# Autodesk Inventor assembly: Gearbox
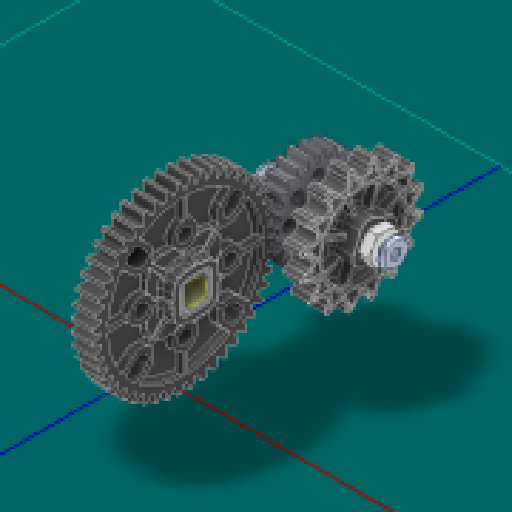
[picture p0: Inventor's stored thumbnail of the model, 512x512]
Saved by Autodesk Inventor 2025 (Build 290162000, 162)
## iProperties
Created: 2024-10-21
Part Number: Gearbox
Document SubType Name: Assembly
Designer: averey
Author: averey
## Documents named in this file (12)
- C:\Users\avere\VEX\High Stakes\CAD\V2\Intake\Gearbox.iam
- Gearbox Left.iam
- C:\Users\avere\VEX\High Stakes\CAD\ROBOPROS-CAD-Inventor\Motion\Sprockets\6P Sprocket\6P 16T Sprocket, No Insert.iam
- C:\Users\avere\VEX\High Stakes\CAD\V2\Intake\Custom Parts\Gearbox Gusset.ipt
- C:\Users\avere\VEX\High Stakes\CAD\ROBOPROS-CAD-Inventor\Structure\Hardware\Nut Nylon\Nut Nylon - White.ipt
- C:\Users\avere\VEX\High Stakes\CAD\ROBOPROS-CAD-Inventor\Structure\Hardware\Nut Nylon.ipt
- C:\Users\avere\VEX\High Stakes\CAD\ROBOPROS-CAD-Inventor\Structure\Hardware\Nut Thin Nylock.ipt
- C:\Users\avere\VEX\High Stakes\CAD\ROBOPROS-CAD-Inventor\Structure\Hardware\Screw Steel - Star\SScrew Star Smooth 1.500.ipt
- C:\Users\avere\VEX\High Stakes\CAD\ROBOPROS-CAD-Inventor\Structure\Hardware\Screw Steel - Star.ipt
- C:\Users\avere\VEX\High Stakes\CAD\ROBOPROS-CAD-Inventor\Motion\Sprockets\6P Sprocket.iam
- C:\Users\avere\VEX\High Stakes\CAD\ROBOPROS-CAD-Inventor\Modified Parts\Half Cut HS 24T Gear, No Insert.ipt
- C:\Users\avere\VEX\High Stakes\CAD\ROBOPROS-CAD-Inventor\Modified Parts\Equal Half Cut HS 48T Gear, No Insert.ipt
## Components (7 placed, 7 different names)
1. 6P 16T Sprocket, No Insert:1 [sub-assembly] — Insert:4
2. Gearbox Gusset:1 — Mate:2, Mate:3, Mate:4, Insert:5, Insert:9, Insert:10
3. Nut Nylon - White:1 — Insert:4, Insert:6
4. Nut Thin Nylock:1 — Insert:5
5. SScrew Star Smooth 1.500:1 — Insert:6
6. Half Cut HS 24T Gear, No Insert:1 — Insert:9
7. Equal Half Cut HS 48T Gear, No Insert:1 — Insert:10
## Relationships (8: Insert 5, Mate 3)
- Mate:2: Gearbox Gusset:1
- Mate:3: Gearbox Gusset:1
- Mate:4: Gearbox Gusset:1
- Insert:4: 6P 16T Sprocket, No Insert:1 ↔ Nut Nylon - White:1
- Insert:5: Gearbox Gusset:1 ↔ Nut Thin Nylock:1
- Insert:6 (1.5875 mm): Nut Nylon - White:1 ↔ SScrew Star Smooth 1.500:1
- Insert:9: Gearbox Gusset:1 ↔ Half Cut HS 24T Gear, No Insert:1
- Insert:10: Gearbox Gusset:1 ↔ Equal Half Cut HS 48T Gear, No Insert:1
